# Autodesk Inventor assembly: FullView
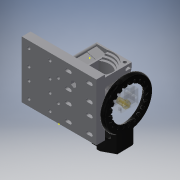
[picture p0: Inventor's stored thumbnail of the model, 180x180]
Saved by Autodesk Inventor 2019 (Build 230136000, 136)
## iProperties
Created: 2018-06-29
Part Number: FullView
Material: Ogólny
Document SubType Name: Assembly
Designer: Kamil
Author: Kamil
## Documents named in this file (6)
- D:\Git\3DPrinting\E3DExtruderHolder\FullView.iam
- D:\Git\3DPrinting\E3DExtruderHolder\ExtruderHolder.ipt
- D:\Git\3DPrinting\E3DExtruderHolder\ExtruderCooler.ipt
- D:\Git\3DPrinting\E3DExtruderHolder\ExtruderClamp.ipt
- C:\Users\Kamil\Desktop\ED3V6.iam
- C:\Users\Kamil\Desktop\FanV2_Shorter.ipt
## Components (5 placed, 5 different names)
1. ExtruderCooler:1
2. ExtruderClamp:1 — Walcowe:1
3. ExtruderHolder:1 — Walcowe:1, Obrotowe:1
4. FanV2_Shorter:1
5. ED3V6:2 [sub-assembly] — Obrotowe:1
## Relationships (2: CylindricalJoint 1, RevoluteJoint 1)
- Walcowe:1 [CylindricalJoint]: ExtruderClamp:1 ↔ ExtruderHolder:1
- Obrotowe:1 [RevoluteJoint]: ExtruderHolder:1 ↔ ED3V6:2
